# Autodesk Inventor assembly: 1400-00 PopCornMachine
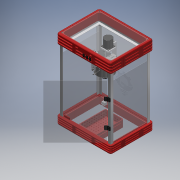
[picture p0: Inventor's stored thumbnail of the model, 180x180]
Saved by Autodesk Inventor 2017 (Build 210142000, 142)
## iProperties
Company: FABLAB Frecnhmakers
Part Number: 1400-00 PopCornMachine
Project: 1400-PopCorn Machine
Material: Générique
Catalog Web Link: http://frenchmakers.com/
Document SubType Name: Assembly
Designer: Adrien MARY
Author: Adrien MARY
## Documents named in this file (43)
- W:\Professionnel\Conception FABLAB\1400 Popcorn Machine\1400-00 PopCornMachine.iam
- W:\Professionnel\Conception FABLAB\1400 Popcorn Machine\1400-06 Profilé\1400-06-03 Profilé vertical.ipt
- W:\Professionnel\Conception FABLAB\1400 Popcorn Machine\1400-04 Plaques\1400-04-02 Plaque superieur.ipt
- W:\Professionnel\Conception FABLAB\1400 Popcorn Machine\1400-06 Profilé\1400-06-01 Profilé superieur cote.ipt
- W:\Professionnel\Conception FABLAB\1400 Popcorn Machine\1400-06 Profilé\1400-06-02 Profilé superieur face.ipt
- W:\Professionnel\Conception FABLAB\1400 Popcorn Machine\1400-04 Plaques\1400-04-05 Plaque support.ipt
- W:\Professionnel\Conception FABLAB\1400 Popcorn Machine\1400-07 Electronique\1400-07-01 Moteur.ipt
- W:\Professionnel\Conception FABLAB\1400 Popcorn Machine\1400-08 Fixation\1400-08-01 Bras.ipt
- W:\Professionnel\Conception FABLAB\1400 Popcorn Machine\1400-01 Casserole\1400-01-00 Casserole.iam
- W:\Professionnel\Conception FABLAB\1400 Popcorn Machine\1400-08 Fixation\1400-08-02 Butee.ipt
- W:\Professionnel\Conception FABLAB\1400 Popcorn Machine\1400-90 Centre de contenu\fr-FR\ISO 4762(2)\ISO 4762 - M4 x 20ISO.ipt
- W:\Professionnel\Conception FABLAB\1400 Popcorn Machine\1400-08 Fixation\1400-08-03 Engrenage Moteur.ipt
- W:\Professionnel\Conception FABLAB\1400 Popcorn Machine\1400-90 Centre de contenu\fr-FR\ISO 4762(2)\ISO 4762 - M3 x 12ISO.ipt
- W:\Professionnel\Conception FABLAB\1400 Popcorn Machine\1400-90 Centre de contenu\fr-FR\ISO 4032(2)\ISO 4032 - M3 - ISO.ipt
- W:\Professionnel\Conception FABLAB\1400 Popcorn Machine\1400-90 Centre de contenu\fr-FR\ISO 4762(2)\ISO 4762 - M5 x 20ISO.ipt
- W:\Professionnel\Conception FABLAB\1400 Popcorn Machine\1400-90 Centre de contenu\fr-FR\ISO 4032(2)\ISO 4032 - M5 - ISO.ipt
- W:\Professionnel\Conception FABLAB\1400 Popcorn Machine\1400-04 Plaques\1400-04-03 Plaque cote.ipt
- W:\Professionnel\Conception FABLAB\1400 Popcorn Machine\1400-04 Plaques\1400-04-04 Plaque fond.ipt
- W:\Professionnel\Conception FABLAB\1400 Popcorn Machine\1400-05 Charniere\1400-05-00 Charniere.iam
- W:\Professionnel\Conception FABLAB\1400 Popcorn Machine\1400-04 Plaques\1400-04-06 Porte.ipt
- W:\Professionnel\Conception FABLAB\1400 Popcorn Machine\1400-04 Plaques\1400-04-01 Plaque inferieur.ipt
- W:\Professionnel\Conception FABLAB\1400 Popcorn Machine\1400-02 Partie inferieur\1400-02-02 Coins A.ipt
- W:\Professionnel\Conception FABLAB\1400 Popcorn Machine\1400-02 Partie inferieur\1400-02-03 Coins B.ipt
- W:\Professionnel\Conception FABLAB\1400 Popcorn Machine\1400-02 Partie inferieur\1400-02-04 Coins C.ipt
- W:\Professionnel\Conception FABLAB\1400 Popcorn Machine\1400-02 Partie inferieur\1400-02-05 Coins D.ipt
- W:\Professionnel\Conception FABLAB\1400 Popcorn Machine\1400-02 Partie inferieur\1400-02-06 Tirroir.ipt
- W:\Professionnel\Conception FABLAB\1400 Popcorn Machine\1400-02 Partie inferieur\1400-02-07 Arriere.ipt
- W:\Professionnel\Conception FABLAB\1400 Popcorn Machine\1400-02 Partie inferieur\1400-02-08 Cote A.ipt
- W:\Professionnel\Conception FABLAB\1400 Popcorn Machine\1400-02 Partie inferieur\1400-02-09 Cote B.ipt
- W:\Professionnel\Conception FABLAB\1400 Popcorn Machine\1400-07 Electronique\1400-07-02 Plug alimentaion.ipt
- W:\Professionnel\Conception FABLAB\1400 Popcorn Machine\1400-90 Centre de contenu\fr-FR\ISO 10642(1)\ISO 10642 - M3 x  25.ipt
- W:\Professionnel\Conception FABLAB\1400 Popcorn Machine\1400-01 Casserole\1400-01-20 Axe.iam
- W:\Professionnel\Conception FABLAB\1400 Popcorn Machine\1400-03 Partie superieur\1400-03-02 Coins E.ipt
- W:\Professionnel\Conception FABLAB\1400 Popcorn Machine\1400-03 Partie superieur\1400-03-03 Coins F.ipt
- W:\Professionnel\Conception FABLAB\1400 Popcorn Machine\1400-03 Partie superieur\1400-03-04 Coins G.ipt
- W:\Professionnel\Conception FABLAB\1400 Popcorn Machine\1400-03 Partie superieur\1400-03-05 Coins H.ipt
- W:\Professionnel\Conception FABLAB\1400 Popcorn Machine\1400-03 Partie superieur\1400-03-06 Avant.ipt
- W:\Professionnel\Conception FABLAB\1400 Popcorn Machine\1400-03 Partie superieur\1400-03-07 Arriere.ipt
- W:\Professionnel\Conception FABLAB\1400 Popcorn Machine\1400-03 Partie superieur\1400-03-08 Cote C.ipt
- W:\Professionnel\Conception FABLAB\1400 Popcorn Machine\1400-03 Partie superieur\1400-03-09 Cote D.ipt
- W:\Professionnel\Conception FABLAB\1400 Popcorn Machine\1400-07 Electronique\1400-07-03 Bonton.ipt
- W:\Professionnel\Conception FABLAB\1400 Popcorn Machine\1400-06 Profilé\1400-06-04 Profilé vertical chaniere.ipt
- W:\Professionnel\Conception FABLAB\1400 Popcorn Machine\1400-90 Centre de contenu\fr-FR\ISO 10642(1)\ISO 10642 - M5 x  12.ipt
## Components (82 placed, 42 different names)
1. 1400-01-20 Axe:1 [sub-assembly] — Placage:86, Affleurement:97, Rotation:1
2. 1400-01-00 Casserole:1 [sub-assembly] — Placage:30, Affleurement:14, Angle:1, Placage:86
3. 1400-02-02 Coins A:1 — Affleurement:79, Affleurement:80, Affleurement:88, Placage:69, Placage:70, Placage:71, Logement:5, Angle:3, Angle:4, Placage:83
4. 1400-02-03 Coins B:1 — Affleurement:72, Affleurement:78, Affleurement:89, Placage:75, Placage:77, Placage:78
5. 1400-02-04 Coins C:1 — Affleurement:73, Affleurement:81, Affleurement:90, Ouverture_tirroir, Placage:74
6. 1400-02-05 Coins D:1 — Affleurement:74, Affleurement:82, Affleurement:91, Placage:82, Placage:84
7. 1400-02-06 Tirroir:1 — Affleurement:75, Affleurement:83, Ouverture_tirroir
8. 1400-02-07 Arriere:1 — Affleurement:76, Affleurement:84, Affleurement:93, Placage:76
9. 1400-02-08 Cote A:1 — Affleurement:77, Affleurement:85, Affleurement:94, Placage:81
10. 1400-02-09 Cote B:1 — Affleurement:87, Affleurement:86, Affleurement:95, Placage:79, Placage:80
11. 1400-03-02 Coins E:1 — Affleurement:98, Placage:88, Affleurement:113, Placage:96, Placage:97, Placage:98, Placage:108
12. 1400-03-03 Coins F:1 — Affleurement:99, Placage:89, Affleurement:112, Affleurement:113
13. 1400-03-04 Coins G:1 — Affleurement:100, Placage:90, Affleurement:111, Affleurement:112
14. 1400-03-05 Coins H:1 — Affleurement:101, Placage:91, Affleurement:110, Affleurement:111, Placage:99
15. 1400-03-06 Avant:1 — Affleurement:102, Placage:92, Affleurement:109, Affleurement:110, Placage:100, Placage:101, Placage:102
16. 1400-03-07 Arriere:1 — Affleurement:103, Placage:93, Affleurement:107, Affleurement:108, Affleurement:109
17. 1400-03-08 Cote C:1 — Affleurement:104, Placage:94, Affleurement:106, Affleurement:107, Affleurement:108
18. 1400-03-09 Cote D:1 — Affleurement:105, Placage:95, Affleurement:106
19. 1400-04-01 Plaque inferieur:1 — Affleurement:70, Affleurement:71
20. 1400-04-02 Plaque superieur:1 — Placage:57, Placage:58, Placage:59, Placage:60, Placage:61, Placage:97, Placage:98, Placage:99
21. 1400-04-03 Plaque cote:2 — Affleurement:24, Affleurement:25, Placage:79, Placage:80
22. 1400-04-03 Plaque cote:1 — Affleurement:24, Affleurement:25, Placage:54, Placage:81
23. 1400-04-04 Plaque fond:1 — Affleurement:26, Placage:75, Placage:76
24. 1400-04-05 Plaque support:1 — Placage:21, Affleurement:11, Affleurement:12, Placage:22, Placage:23, Placage:24, Placage:25, Placage:26, Placage:27, Placage:28, Placage:29, Placage:31, Placage:32, Placage:33, Placage:46
25. 1400-04-06 Porte:1 — Placage:84, Placage:106, Placage:107, Logement:14, Logement:15, Logement:16, Logement:17
26. 1400-05-00 Charniere:2 [sub-assembly] — Affleurement:120, Placage:103, Affleurement:121, Placage:105, Placage:106, Placage:107, Logement:6, Logement:7, Logement:8, Logement:9
27. 1400-05-00 Charniere:1 [sub-assembly] — Affleurement:120, Affleurement:121, Placage:104, Logement:10, Logement:11, Logement:12, Logement:13
28. 1400-06-02 Profilé superieur face:2 — Placage:14, Placage:15, Placage:16, Placage:17, Placage:18, Affleurement:122
29. 1400-06-01 Profilé superieur cote:2 — Placage:16, Placage:17, Placage:19, Placage:21, Affleurement:122, Affleurement:123, Placage:108
30. 1400-06-02 Profilé superieur face:1 — Placage:12, Placage:13, Affleurement:123, Affleurement:124
31. 1400-06-01 Profilé superieur cote:1 — Placage:12, Placage:13, Placage:14, Placage:15, Affleurement:124
32. 1400-06-03 Profilé vertical:4 — Affleurement:2, Affleurement:3, Affleurement:4, Affleurement:6, Placage:77, Placage:78
33. 1400-06-03 Profilé vertical:3 — Affleurement:3, Affleurement:4, Affleurement:5, Placage:74, Placage:83, Placage:96
34. 1400-06-03 Profilé vertical:2 — Affleurement:1, Affleurement:5, Affleurement:7, Placage:18, Placage:19
35. 1400-06-04 Profilé vertical chaniere:1 — Affleurement:1, Affleurement:2, Affleurement:6, Affleurement:7, Placage:82, Placage:103, Placage:104, Placage:105, Logement:18, Logement:19, Logement:20, Logement:21
36. 1400-07-01 Moteur:1 — Placage:22, Placage:23, Placage:24, Placage:39, Placage:87
37. 1400-07-02 Plug alimentaion:1 — Placage:69, Placage:70, Placage:71, Logement:3, Logement:4
38. 1400-07-03 Bonton:1 — Affleurement:114, Affleurement:116, Placage:100, Placage:101, Placage:102, Affleurement:119
39. 1400-07-03 Bonton:2 — Affleurement:114, Affleurement:115, Affleurement:116, Affleurement:117, Affleurement:118, Affleurement:119
40. 1400-07-03 Bonton:3 — Affleurement:115, Affleurement:117, Affleurement:118
41. 1400-08-01 Bras:1 — Affleurement:13, Placage:25, Placage:26, Placage:27, Placage:44, Placage:45
42. 1400-08-01 Bras:2 — Affleurement:13, Placage:28, Placage:29, Placage:30, Placage:41, Placage:42, Placage:43
43. 1400-08-02 Butee:1 — Placage:31, Placage:32, Placage:33, Placage:34, Placage:35, Placage:36, Placage:37, Placage:38
44. 1400-08-03 Engrenage Moteur:1 — Placage:39, Logement:1, Logement:2, Angle:2, Affleurement:97, Placage:87, Rotation_moteur, Rotation:1
45. ISO 4762 M3 x 12:2 — Affleurement:27, Affleurement:28, Placage:57, Placage:58
46. ISO 4762 M3 x 12:3 — Affleurement:27, Placage:59
47. ISO 4762 M3 x 12:4 — Affleurement:28, Affleurement:29, Placage:60
48. ISO 4762 M3 x 12:5 — Affleurement:29, Placage:61
49. ISO 10642 M5 x  12:1 — Logement:7
50. ISO 10642 M5 x  12:2 — Logement:8
51. ISO 10642 M5 x  12:3 — Logement:12
52. ISO 10642 M5 x  12:4 — Logement:10
53. ISO 10642 M5 x  12:5 — Logement:9
54. ISO 10642 M5 x  12:6 — Logement:13
55. ISO 10642 M5 x  12:7 — Logement:11
56. ISO 10642 M5 x  12:8 — Logement:6
57. ISO 4032 M5:5 — Logement:14
58. ISO 4032 M5:6 — Logement:17
59. ISO 4032 M5:7 — Logement:18
60. ISO 4032 M5:8 — Logement:20
61. ISO 4032 M5:9 — Logement:19
62. ISO 4032 M5:10 — Logement:15
63. ISO 4032 M5:11 — Logement:16
64. ISO 4032 M5:12 — Logement:21
65. ISO 4762 M4 x 20:1 — Affleurement:17, Placage:36
66. ISO 4762 M4 x 20:2 — Affleurement:16, Placage:38
67. ISO 4762 M4 x 20:3 — Affleurement:15, Affleurement:16, Affleurement:17, Placage:37
68. ISO 4762 M4 x 20:4 — Affleurement:15, Placage:34, Placage:35
69. ISO 10642 M3 x  25:1 — Logement:3, Placage:72
70. ISO 10642 M3 x  25:2 — Logement:4
71. ISO 4032 M3:2 — Affleurement:96, Logement:5, Angle:3
72. ISO 4032 M3:3 — Affleurement:96, Placage:72, Angle:4
73. ISO 4762 M5 x 20:1 — Affleurement:18, Placage:41, Placage:42, Placage:47
74. ISO 4762 M5 x 20:2 — Affleurement:18, Affleurement:19, Placage:43, Placage:48
75. ISO 4762 M5 x 20:3 — Affleurement:19, Affleurement:20, Placage:44, Placage:49
76. ISO 4762 M5 x 20:4 — Affleurement:20, Placage:45, Placage:50
77. ISO 4032 M5:1 — Affleurement:21, Placage:49
78. ISO 4032 M5:2 — Affleurement:23, Placage:46, Placage:47
79. ISO 4032 M5:3 — Affleurement:22, Affleurement:23, Placage:48
80. ISO 4032 M5:4 — Affleurement:21, Affleurement:22, Placage:50
81. ISO 4032 M3:1 — Logement:2, Angle:2
82. ISO 4762 M3 x 12:1 — Logement:1
## Relationships (189: Mate 82, Flush 80, Insert 21, Angle 5, RelateRotation 1)
- Affleurement:1 [Flush]: 1400-06-03 Profilé vertical:2 ↔ 1400-06-04 Profilé vertical chaniere:1
- Affleurement:2 [Flush]: 1400-06-03 Profilé vertical:4 ↔ 1400-06-04 Profilé vertical chaniere:1
- Affleurement:3 [Flush]: 1400-06-03 Profilé vertical:4 ↔ 1400-06-03 Profilé vertical:3
- Affleurement:4 [Flush]: 1400-06-03 Profilé vertical:4 ↔ 1400-06-03 Profilé vertical:3
- Affleurement:5 [Flush]: 1400-06-03 Profilé vertical:3 ↔ 1400-06-03 Profilé vertical:2
- Affleurement:6 [Flush]: 1400-06-03 Profilé vertical:4 ↔ 1400-06-04 Profilé vertical chaniere:1
- Affleurement:7 [Flush]: 1400-06-03 Profilé vertical:2 ↔ 1400-06-04 Profilé vertical chaniere:1
- Placage:12 [Mate]: 1400-06-02 Profilé superieur face:1 ↔ 1400-06-01 Profilé superieur cote:1
- Placage:13 [Mate]: 1400-06-02 Profilé superieur face:1 ↔ 1400-06-01 Profilé superieur cote:1
- Placage:14 [Mate]: 1400-06-02 Profilé superieur face:2 ↔ 1400-06-01 Profilé superieur cote:1
- Placage:15 [Mate]: 1400-06-02 Profilé superieur face:2 ↔ 1400-06-01 Profilé superieur cote:1
- Placage:16 [Mate]: 1400-06-02 Profilé superieur face:2 ↔ 1400-06-01 Profilé superieur cote:2
- Placage:17 [Mate]: 1400-06-02 Profilé superieur face:2 ↔ 1400-06-01 Profilé superieur cote:2
- Placage:18 [Mate]: 1400-06-02 Profilé superieur face:2 ↔ 1400-06-03 Profilé vertical:2
- Placage:19 [Mate]: 1400-06-01 Profilé superieur cote:2 ↔ 1400-06-03 Profilé vertical:2
- Placage:21 [Mate]: 1400-04-05 Plaque support:1 ↔ 1400-06-01 Profilé superieur cote:2
- Affleurement:11 [Flush]: 1400-04-05 Plaque support:1
- Affleurement:12 [Flush]: 1400-04-05 Plaque support:1
- Placage:22 [Mate]: 1400-04-05 Plaque support:1 ↔ 1400-07-01 Moteur:1
- Placage:23 [Mate]: 1400-04-05 Plaque support:1 ↔ 1400-07-01 Moteur:1
- Placage:24 [Mate]: 1400-04-05 Plaque support:1 ↔ 1400-07-01 Moteur:1
- Affleurement:13 [Flush]: 1400-08-01 Bras:1 ↔ 1400-08-01 Bras:2
- Placage:25 [Mate]: 1400-04-05 Plaque support:1 ↔ 1400-08-01 Bras:1
- Placage:26 [Mate]: 1400-04-05 Plaque support:1 ↔ 1400-08-01 Bras:1
- Placage:27 [Mate]: 1400-04-05 Plaque support:1 ↔ 1400-08-01 Bras:1
- Placage:28 [Mate]: 1400-04-05 Plaque support:1 ↔ 1400-08-01 Bras:2
- Placage:29 [Mate]: 1400-04-05 Plaque support:1 ↔ 1400-08-01 Bras:2
- Placage:30 [Mate]: 1400-01-00 Casserole:1 ↔ 1400-08-01 Bras:2
- Affleurement:14 [Flush]: 1400-01-00 Casserole:1
- Angle:1 (180 deg): 1400-01-00 Casserole:1
- Placage:31 [Mate]: 1400-04-05 Plaque support:1 ↔ 1400-08-02 Butee:1
- Placage:32 [Mate]: 1400-04-05 Plaque support:1 ↔ 1400-08-02 Butee:1
- Placage:33 [Mate]: 1400-04-05 Plaque support:1 ↔ 1400-08-02 Butee:1
- Affleurement:15 [Flush]: ISO 4762 M4 x 20:3 ↔ ISO 4762 M4 x 20:4
- Affleurement:16 [Flush]: ISO 4762 M4 x 20:2 ↔ ISO 4762 M4 x 20:3
- Affleurement:17 [Flush]: ISO 4762 M4 x 20:1 ↔ ISO 4762 M4 x 20:3
- Placage:34 [Mate]: 1400-08-02 Butee:1 ↔ ISO 4762 M4 x 20:4
- Placage:35 [Mate]: 1400-08-02 Butee:1 ↔ ISO 4762 M4 x 20:4
- Placage:36 [Mate]: 1400-08-02 Butee:1 ↔ ISO 4762 M4 x 20:1
- Placage:37 [Mate]: 1400-08-02 Butee:1 ↔ ISO 4762 M4 x 20:3
- Placage:38 [Mate]: 1400-08-02 Butee:1 ↔ ISO 4762 M4 x 20:2
- Placage:39 [Mate]: 1400-07-01 Moteur:1 ↔ 1400-08-03 Engrenage Moteur:1
- Logement:1 [Insert]: 1400-08-03 Engrenage Moteur:1 ↔ ISO 4762 M3 x 12:1
- Logement:2 [Insert]: 1400-08-03 Engrenage Moteur:1 ↔ ISO 4032 M3:1
- Angle:2 (0 deg): 1400-08-03 Engrenage Moteur:1 ↔ ISO 4032 M3:1
- Affleurement:18 [Flush]: ISO 4762 M5 x 20:1 ↔ ISO 4762 M5 x 20:2
- Affleurement:19 [Flush]: ISO 4762 M5 x 20:2 ↔ ISO 4762 M5 x 20:3
- Affleurement:20 [Flush]: ISO 4762 M5 x 20:3 ↔ ISO 4762 M5 x 20:4
- Placage:41 [Mate]: 1400-08-01 Bras:2 ↔ ISO 4762 M5 x 20:1
- Placage:42 [Mate]: 1400-08-01 Bras:2 ↔ ISO 4762 M5 x 20:1
- Placage:43 [Mate]: 1400-08-01 Bras:2 ↔ ISO 4762 M5 x 20:2
- Placage:44 [Mate]: 1400-08-01 Bras:1 ↔ ISO 4762 M5 x 20:3
- Placage:45 [Mate]: 1400-08-01 Bras:1 ↔ ISO 4762 M5 x 20:4
- Affleurement:21 [Flush]: ISO 4032 M5:1 ↔ ISO 4032 M5:4
- Affleurement:22 [Flush]: ISO 4032 M5:3 ↔ ISO 4032 M5:4
- Affleurement:23 [Flush]: ISO 4032 M5:2 ↔ ISO 4032 M5:3
- Placage:46 [Mate]: 1400-04-05 Plaque support:1 ↔ ISO 4032 M5:2
- Placage:47 [Mate]: ISO 4762 M5 x 20:1 ↔ ISO 4032 M5:2
- Placage:48 [Mate]: ISO 4762 M5 x 20:2 ↔ ISO 4032 M5:3
- Placage:49 [Mate]: ISO 4762 M5 x 20:3 ↔ ISO 4032 M5:1
- Placage:50 [Mate]: ISO 4762 M5 x 20:4 ↔ ISO 4032 M5:4
- Affleurement:24 [Flush]: 1400-04-03 Plaque cote:2 ↔ 1400-04-03 Plaque cote:1
- Affleurement:25 [Flush]: 1400-04-03 Plaque cote:2 ↔ 1400-04-03 Plaque cote:1
- Placage:54 [Mate]: 1400-04-03 Plaque cote:1
- Affleurement:26 [Flush]: 1400-04-04 Plaque fond:1
- Affleurement:27 [Flush]: ISO 4762 M3 x 12:2 ↔ ISO 4762 M3 x 12:3
- Affleurement:28 [Flush]: ISO 4762 M3 x 12:2 ↔ ISO 4762 M3 x 12:4
- Affleurement:29 [Flush]: ISO 4762 M3 x 12:4 ↔ ISO 4762 M3 x 12:5
- Placage:57 [Mate]: 1400-04-02 Plaque superieur:1 ↔ ISO 4762 M3 x 12:2
- Placage:58 [Mate]: 1400-04-02 Plaque superieur:1 ↔ ISO 4762 M3 x 12:2
- Placage:59 [Mate]: 1400-04-02 Plaque superieur:1 ↔ ISO 4762 M3 x 12:3
- Placage:60 [Mate]: 1400-04-02 Plaque superieur:1 ↔ ISO 4762 M3 x 12:4
- Placage:61 [Mate]: 1400-04-02 Plaque superieur:1 ↔ ISO 4762 M3 x 12:5
- Affleurement:70 [Flush]: 1400-04-01 Plaque inferieur:1
- Affleurement:71 [Flush]: 1400-04-01 Plaque inferieur:1
- Affleurement:72 [Flush]: 1400-02-03 Coins B:1
- Affleurement:73 [Flush]: 1400-02-04 Coins C:1
- Affleurement:74 [Flush]: 1400-02-05 Coins D:1
- Affleurement:75 [Flush]: 1400-02-06 Tirroir:1
- Affleurement:76 [Flush]: 1400-02-07 Arriere:1
- Affleurement:77 [Flush]: 1400-02-08 Cote A:1
- Affleurement:87 [Flush]: 1400-02-09 Cote B:1
- Affleurement:78 [Flush]: 1400-02-03 Coins B:1
- Affleurement:79 [Flush]: 1400-02-02 Coins A:1
- Affleurement:80 [Flush]: 1400-02-02 Coins A:1
- Affleurement:81 [Flush]: 1400-02-04 Coins C:1
- Affleurement:82 [Flush]: 1400-02-05 Coins D:1
- Affleurement:83 [Flush]: 1400-02-06 Tirroir:1
- Affleurement:84 [Flush]: 1400-02-07 Arriere:1
- Affleurement:85 [Flush]: 1400-02-08 Cote A:1
- Affleurement:86 [Flush]: 1400-02-09 Cote B:1
- Affleurement:88 [Flush]: 1400-02-02 Coins A:1
- Affleurement:89 [Flush]: 1400-02-03 Coins B:1
- Affleurement:90 [Flush]: 1400-02-04 Coins C:1
- Affleurement:91 [Flush]: 1400-02-05 Coins D:1
- Affleurement:93 [Flush]: 1400-02-07 Arriere:1
- Affleurement:94 [Flush]: 1400-02-08 Cote A:1
- Affleurement:95 [Flush]: 1400-02-09 Cote B:1
- Placage:69 [Mate]: 1400-02-02 Coins A:1 ↔ 1400-07-02 Plug alimentaion:1
- Placage:70 [Mate]: 1400-02-02 Coins A:1 ↔ 1400-07-02 Plug alimentaion:1
- Placage:71 [Mate]: 1400-02-02 Coins A:1 ↔ 1400-07-02 Plug alimentaion:1
- Logement:3 [Insert]: 1400-07-02 Plug alimentaion:1 ↔ ISO 10642 M3 x  25:1
- Logement:4 [Insert]: 1400-07-02 Plug alimentaion:1 ↔ ISO 10642 M3 x  25:2
- Affleurement:96 [Flush]: ISO 4032 M3:2 ↔ ISO 4032 M3:3
- Logement:5 [Insert]: 1400-02-02 Coins A:1 ↔ ISO 4032 M3:2
- Angle:3 (0 deg): 1400-02-02 Coins A:1 ↔ ISO 4032 M3:2
- Placage:72 [Mate]: ISO 10642 M3 x  25:1 ↔ ISO 4032 M3:3
- Angle:4 (0 deg): 1400-02-02 Coins A:1 ↔ ISO 4032 M3:3
- Ouverture_tirroir [Mate]: 1400-02-04 Coins C:1 ↔ 1400-02-06 Tirroir:1
- Placage:74 [Mate]: 1400-02-04 Coins C:1 ↔ 1400-06-03 Profilé vertical:3
- Placage:75 [Mate]: 1400-02-03 Coins B:1 ↔ 1400-04-04 Plaque fond:1
- Placage:76 [Mate]: 1400-02-07 Arriere:1 ↔ 1400-04-04 Plaque fond:1
- Placage:77 [Mate]: 1400-02-03 Coins B:1 ↔ 1400-06-03 Profilé vertical:4
- Placage:78 [Mate]: 1400-02-03 Coins B:1 ↔ 1400-06-03 Profilé vertical:4
- Placage:79 [Mate]: 1400-02-09 Cote B:1 ↔ 1400-04-03 Plaque cote:2
- Placage:80 [Mate]: 1400-02-09 Cote B:1 ↔ 1400-04-03 Plaque cote:2
- Placage:81 [Mate]: 1400-02-08 Cote A:1 ↔ 1400-04-03 Plaque cote:1
- Placage:82 [Mate]: 1400-02-05 Coins D:1 ↔ 1400-06-04 Profilé vertical chaniere:1
- Placage:83 [Mate]: 1400-02-02 Coins A:1 ↔ 1400-06-03 Profilé vertical:3
- Placage:84 [Mate] (1 mm): 1400-02-05 Coins D:1 ↔ 1400-04-06 Porte:1
- Placage:86 [Mate]: 1400-01-20 Axe:1 ↔ 1400-01-00 Casserole:1
- Affleurement:97 [Flush]: 1400-01-20 Axe:1 ↔ 1400-08-03 Engrenage Moteur:1
- Placage:87 [Mate] (-8 mm): 1400-07-01 Moteur:1 ↔ 1400-08-03 Engrenage Moteur:1
- Rotation_moteur [Angle] (0 deg): 1400-08-03 Engrenage Moteur:1
- Rotation:1 [RelateRotation] (1 ul): 1400-01-20 Axe:1 ↔ 1400-08-03 Engrenage Moteur:1
- Affleurement:98 [Flush]: 1400-03-02 Coins E:1
- Affleurement:99 [Flush]: 1400-03-03 Coins F:1
- Affleurement:100 [Flush]: 1400-03-04 Coins G:1
- Affleurement:101 [Flush]: 1400-03-05 Coins H:1
- Affleurement:102 [Flush]: 1400-03-06 Avant:1
- Affleurement:103 [Flush]: 1400-03-07 Arriere:1
- Affleurement:104 [Flush]: 1400-03-08 Cote C:1
- Affleurement:105 [Flush]: 1400-03-09 Cote D:1
- Placage:88 [Mate]: 1400-03-02 Coins E:1
- Placage:89 [Mate]: 1400-03-03 Coins F:1
- Placage:90 [Mate]: 1400-03-04 Coins G:1
- Placage:91 [Mate]: 1400-03-05 Coins H:1
- Placage:92 [Mate]: 1400-03-06 Avant:1
- Placage:93 [Mate]: 1400-03-07 Arriere:1
- Placage:94 [Mate]: 1400-03-08 Cote C:1
- Placage:95 [Mate]: 1400-03-09 Cote D:1
- Affleurement:106 [Flush]: 1400-03-08 Cote C:1 ↔ 1400-03-09 Cote D:1
- Affleurement:107 [Flush]: 1400-03-07 Arriere:1 ↔ 1400-03-08 Cote C:1
- Affleurement:108 [Flush]: 1400-03-07 Arriere:1 ↔ 1400-03-08 Cote C:1
- Affleurement:109 [Flush]: 1400-03-06 Avant:1 ↔ 1400-03-07 Arriere:1
- Affleurement:110 [Flush]: 1400-03-05 Coins H:1 ↔ 1400-03-06 Avant:1
- Affleurement:111 [Flush]: 1400-03-04 Coins G:1 ↔ 1400-03-05 Coins H:1
- Affleurement:112 [Flush]: 1400-03-03 Coins F:1 ↔ 1400-03-04 Coins G:1
- Affleurement:113 [Flush]: 1400-03-02 Coins E:1 ↔ 1400-03-03 Coins F:1
- Placage:96 [Mate]: 1400-03-02 Coins E:1 ↔ 1400-06-03 Profilé vertical:3
- Placage:97 [Mate]: 1400-03-02 Coins E:1 ↔ 1400-04-02 Plaque superieur:1
- Placage:98 [Mate]: 1400-03-02 Coins E:1 ↔ 1400-04-02 Plaque superieur:1
- Placage:99 [Mate]: 1400-03-05 Coins H:1 ↔ 1400-04-02 Plaque superieur:1
- Affleurement:114 [Flush]: 1400-07-03 Bonton:1 ↔ 1400-07-03 Bonton:2
- Affleurement:115 [Flush]: 1400-07-03 Bonton:2 ↔ 1400-07-03 Bonton:3
- Affleurement:116 [Flush]: 1400-07-03 Bonton:1 ↔ 1400-07-03 Bonton:2
- Affleurement:117 [Flush]: 1400-07-03 Bonton:2 ↔ 1400-07-03 Bonton:3
- Placage:100 [Mate]: 1400-03-06 Avant:1 ↔ 1400-07-03 Bonton:1
- Placage:101 [Mate]: 1400-03-06 Avant:1 ↔ 1400-07-03 Bonton:1
- Placage:102 [Mate]: 1400-03-06 Avant:1 ↔ 1400-07-03 Bonton:1
- Affleurement:118 [Flush] (-25 mm): 1400-07-03 Bonton:2 ↔ 1400-07-03 Bonton:3
- Affleurement:119 [Flush] (25 mm): 1400-07-03 Bonton:1 ↔ 1400-07-03 Bonton:2
- Affleurement:120 [Flush]: 1400-05-00 Charniere:2 ↔ 1400-05-00 Charniere:1
- Placage:103 [Mate]: 1400-05-00 Charniere:2 ↔ 1400-06-04 Profilé vertical chaniere:1
- Affleurement:121 [Flush]: 1400-05-00 Charniere:2 ↔ 1400-05-00 Charniere:1
- Placage:104 [Mate]: 1400-05-00 Charniere:1 ↔ 1400-06-04 Profilé vertical chaniere:1
- Placage:105 [Mate]: 1400-05-00 Charniere:2 ↔ 1400-06-04 Profilé vertical chaniere:1
- Placage:106 [Mate]: 1400-04-06 Porte:1 ↔ 1400-05-00 Charniere:2
- Placage:107 [Mate]: 1400-04-06 Porte:1 ↔ 1400-05-00 Charniere:2
- Affleurement:122 [Flush]: 1400-06-02 Profilé superieur face:2 ↔ 1400-06-01 Profilé superieur cote:2
- Affleurement:123 [Flush]: 1400-06-01 Profilé superieur cote:2 ↔ 1400-06-02 Profilé superieur face:1
- Affleurement:124 [Flush]: 1400-06-02 Profilé superieur face:1 ↔ 1400-06-01 Profilé superieur cote:1
- Placage:108 [Mate]: 1400-03-02 Coins E:1 ↔ 1400-06-01 Profilé superieur cote:2
- Logement:6 [Insert]: 1400-05-00 Charniere:2 ↔ ISO 10642 M5 x  12:8
- Logement:7 [Insert]: 1400-05-00 Charniere:2 ↔ ISO 10642 M5 x  12:1
- Logement:8 [Insert]: 1400-05-00 Charniere:2 ↔ ISO 10642 M5 x  12:2
- Logement:9 [Insert]: 1400-05-00 Charniere:2 ↔ ISO 10642 M5 x  12:5
- Logement:10 [Insert]: 1400-05-00 Charniere:1 ↔ ISO 10642 M5 x  12:4
- Logement:11 [Insert]: 1400-05-00 Charniere:1 ↔ ISO 10642 M5 x  12:7
- Logement:12 [Insert]: 1400-05-00 Charniere:1 ↔ ISO 10642 M5 x  12:3
- Logement:13 [Insert]: 1400-05-00 Charniere:1 ↔ ISO 10642 M5 x  12:6
- Logement:14 [Insert]: 1400-04-06 Porte:1 ↔ ISO 4032 M5:5
- Logement:15 [Insert]: 1400-04-06 Porte:1 ↔ ISO 4032 M5:10
- Logement:16 [Insert]: 1400-04-06 Porte:1 ↔ ISO 4032 M5:11
- Logement:17 [Insert]: 1400-04-06 Porte:1 ↔ ISO 4032 M5:6
- Logement:18 [Insert]: 1400-06-04 Profilé vertical chaniere:1 ↔ ISO 4032 M5:7
- Logement:19 [Insert]: 1400-06-04 Profilé vertical chaniere:1 ↔ ISO 4032 M5:9
- Logement:20 [Insert]: 1400-06-04 Profilé vertical chaniere:1 ↔ ISO 4032 M5:8
- Logement:21 [Insert]: 1400-06-04 Profilé vertical chaniere:1 ↔ ISO 4032 M5:12
## Named parameters: Ouverture_tirroir = 0 mm, Rotation_moteur = 0 deg
